# Autodesk Inventor assembly: Intake
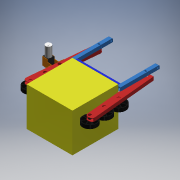
[picture p0: Inventor's stored thumbnail of the model, 180x180]
Saved by Autodesk Inventor 2017 SP1 (Build 210196100, 196)
## iProperties
Created: 2018-01-23
Part Number: Intake
Document SubType Name: Assembly
Designer: Ben
Mass: 2492.9 g
Surface Area: 13580.9 cm^2
Volume: 31878.5 cm^3
Density: 0.0782001 g/cm^3
Author: Ben
## Documents named in this file (9)
- C:\Users\Ben\Desktop\Projects\2018 Robot\Cube Intake\Intake.iam
- C:\Users\Ben\Desktop\Projects\2018 Robot\Cube Intake\arm.ipt
- C:\Users\Ben\Desktop\Projects\2018 Robot\Cube Intake\intake roller.ipt
- C:\Users\Ben\Desktop\Projects\2018 Robot\Cube Lift\cube.ipt
- C:\Users\Ben\Desktop\Projects\2018 Robot\Cube Intake\pivot arm.ipt
- C:\Users\Ben\Desktop\Projects\2018 Robot\Cube Intake\cross brace.ipt
- C:\Users\Ben\Desktop\Projects\2018 Robot\Cube Intake\rest plate.ipt
- C:\Users\Ben\Desktop\Projects\2018 Robot\Cube Intake\micro cim.ipt
- C:\Users\Ben\Desktop\Projects\2018 Robot\Cube Intake\motor mount.ipt
## Components (16 placed, 8 different names)
1. arm:1 — Symmetry:1, Insert:1, Insert:2, Insert:3, Insert:10
2. arm:2 — Symmetry:1, Insert:4, Insert:5, Insert:6, Insert:7, Mate:12, Mate:13, Flush:8, Flush:9
3. intake roller:1 — Insert:2
4. intake roller:2 — Insert:1, Tangent:1
5. intake roller:3 — Insert:6
6. intake roller:4 — Insert:4
7. intake roller:5 — Insert:5
8. intake roller:6 — Insert:3
9. cube:1 — Mate:5, Flush:2, Tangent:1
10. pivot arm:1 — Mate:6, Mate:7, Mate:8, Flush:3, Symmetry:2, Insert:7, Mate:16
11. pivot arm:2 — Mate:8, Flush:3, Symmetry:2, Angle:1, Flush:4, Flush:5, Mate:10, Insert:10
12. cross brace:1 — Flush:4, Flush:5, Mate:10, Mate:11, Flush:6, Mate:16
13. rest plate:1 — Mate:11, Flush:6, Flush:7
14. micro cim:1 — Mate:14, Mate:15, Insert:9
15. motor mount:1 — Mate:12, Mate:14, Flush:8, Insert:9
16. motor mount:2 — Mate:13, Mate:15, Flush:9
## Relationships (32: Mate 11, Insert 9, Flush 8, Symmetry 2, Angle 1, Tangent 1)
- Symmetry:1: arm:1 ↔ arm:2
- Insert:1 (3.175 mm): arm:1 ↔ intake roller:2
- Insert:2 (3.175 mm): arm:1 ↔ intake roller:1
- Insert:3 (3.175 mm): arm:1 ↔ intake roller:6
- Insert:4 (3.175 mm): arm:2 ↔ intake roller:4
- Insert:5 (3.175 mm): arm:2 ↔ intake roller:5
- Insert:6 (3.175 mm): arm:2 ↔ intake roller:3
- Mate:5 (-247.65 mm): cube:1
- Flush:2: cube:1
- Mate:6: pivot arm:1
- Mate:7: pivot arm:1
- Mate:8: pivot arm:1 ↔ pivot arm:2
- Flush:3: pivot arm:1 ↔ pivot arm:2
- Symmetry:2: pivot arm:1 ↔ pivot arm:2
- Insert:7 (1.5875 mm): arm:2 ↔ pivot arm:1
- Angle:1 (0 deg): pivot arm:2
- Tangent:1 (25.4 mm): intake roller:2 ↔ cube:1
- Flush:4: pivot arm:2 ↔ cross brace:1
- Flush:5: pivot arm:2 ↔ cross brace:1
- Mate:10: pivot arm:2 ↔ cross brace:1
- Mate:11: cross brace:1 ↔ rest plate:1
- Flush:6: cross brace:1 ↔ rest plate:1
- Flush:7: rest plate:1
- Mate:12: arm:2 ↔ motor mount:1
- Mate:13: arm:2 ↔ motor mount:2
- Mate:14: micro cim:1 ↔ motor mount:1
- Mate:15: micro cim:1 ↔ motor mount:2
- Flush:8: arm:2 ↔ motor mount:1
- Flush:9: arm:2 ↔ motor mount:2
- Insert:9: micro cim:1 ↔ motor mount:1
- Mate:16: pivot arm:1 ↔ cross brace:1
- Insert:10 (1.5875 mm): arm:1 ↔ pivot arm:2
